# Autodesk Inventor assembly: 50mm Stroke Pneumatic Cylinder.f3d
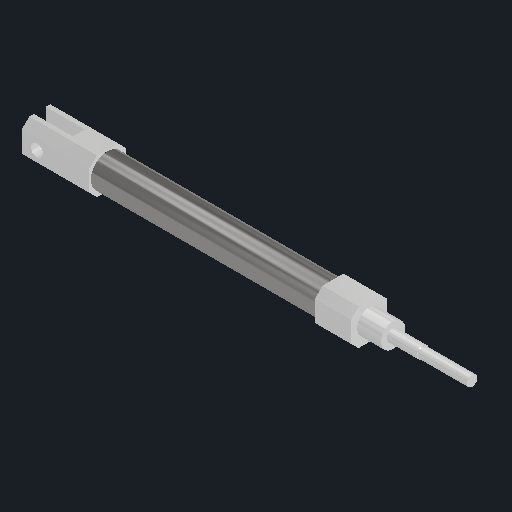
[picture p0: Inventor's stored thumbnail of the model, 512x512]
Saved by Autodesk Inventor 2026.1 (Build 301233000, 233)
## iProperties
Created: 2024-08-07
Part Number: 50mm Stroke Pneumatic Cylinder.f3d
Document SubType Name: Assembly
Designer: chase
Sending System: Autodesk Translation Framework v12.20.1.177
Preprocessor: ST-DEVELOPER v20
Title: 50mm Stroke Pneumatic Cylinder.f3d v1.step
## Documents named in this file (3)
- C:\Users\roejo\OneDrive\Documents\2026WorldChampionRobot\Library\VEX-CAD-Inventor-1.4.2\Motion\Pneumatics\New - V5 Pneumatics\50mm Stroke Pneumatic Cylinder.iam
- C:\Users\roejo\OneDrive\Documents\2026WorldChampionRobot\Library\VEX-CAD-Inventor-1.4.2\Motion\Pneumatics\Reference Parts\Pistons\50mm Stroke Pneumatic Cylinder Body.ipt
- C:\Users\roejo\OneDrive\Documents\2026WorldChampionRobot\Library\VEX-CAD-Inventor-1.4.2\Motion\Pneumatics\Reference Parts\Pistons\50mm Stroke Pneumatic Cylinder Rod.ipt
## Components (2 placed, 2 different names)
1. Component1:1 — Insert:1
2. Component2:1 — Insert:1
## Relationships (1: Insert 1)
- Insert:1: Component1:1 ↔ Component2:1
